# Autodesk Inventor assembly: Donna-Sym2
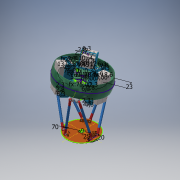
[picture p0: Inventor's stored thumbnail of the model, 180x180]
Saved by Autodesk Inventor 2018.2 (Build 222227000, 227)
## iProperties
Created: 2018-03-01
Part Number: Donna-Sym2
Material: Generisch
Document SubType Name: Assembly
Designer: JochenAlt
Author: JochenAlt
## Documents named in this file (5)
- D:\Projects\Donna\CAD\KST DS215MG\Donna-Sym.iam
- D:\Projects\Donna\CAD\KST DS215MG\Stewart-Sym-Base.iam
- D:\Projects\Donna\CAD\KST DS215MG\Body-Rod-KST215MG.iam
- D:\Projects\Donna\CAD\KST DS215MG\Servo-Arm-20mm-Enhanced-Ball-Joint.iam
- D:\Projects\Donna\CAD\KST DS215MG\Stewart-Body-Sym.iam
## Components (14 placed, 4 different names)
1. Stewart-Sym-Base:1 [sub-assembly] — Passend:1, Passend:2, Passend:3, Passend:4, Passend:5, Passend:6, Passend:7, Passend:8, Passend:9
2. BodyRod-KST215MG:1 [sub-assembly] — Passend:4, Passend:15
3. BodyRod-KST215MG:2 [sub-assembly] — Passend:5, Passend:12
4. BodyRod-KST215MG:3 [sub-assembly] — Passend:6, Passend:27
5. BodyRod-KST215MG:4 [sub-assembly] — Passend:7, Passend:24
6. BodyRod-KST215MG:5 [sub-assembly] — Passend:8, Passend:21
7. BodyRod-KST215MG:6 [sub-assembly] — Passend:9, Passend:18
8. Servo-Arm-20mm-Enhanced-Ball-Joint:1 [sub-assembly] — Passend:22, Passend:23, Passend:24
9. Servo-Arm-20mm-Enhanced-Ball-Joint:2 [sub-assembly] — Passend:10, Passend:11, Passend:12
10. Servo-Arm-20mm-Enhanced-Ball-Joint:3 [sub-assembly] — Passend:19, Passend:20, Passend:21
11. Servo-Arm-20mm-Enhanced-Ball-Joint:4 [sub-assembly] — Passend:25, Passend:26, Passend:27
12. Servo-Arm-20mm-Enhanced-Ball-Joint:5 [sub-assembly] — Passend:16, Passend:17, Passend:18
13. Servo-Arm-20mm-Enhanced-Ball-Joint:6 [sub-assembly] — Passend:13, Passend:14, Passend:15
14. Stewart-Bosy-Sym:1 [sub-assembly] — Passend:10, Passend:11, Passend:13, Passend:14, Passend:16, Passend:17, Passend:19, Passend:20, Passend:22, Passend:23, Passend:25, Passend:26
## Relationships (27: Mate 27)
- Passend:1 [Mate]: Stewart-Sym-Base:1
- Passend:2 [Mate]: Stewart-Sym-Base:1
- Passend:3 [Mate]: Stewart-Sym-Base:1
- Passend:4 [Mate]: Stewart-Sym-Base:1 ↔ BodyRod-KST215MG:1
- Passend:5 [Mate]: Stewart-Sym-Base:1 ↔ BodyRod-KST215MG:2
- Passend:6 [Mate]: Stewart-Sym-Base:1 ↔ BodyRod-KST215MG:3
- Passend:7 [Mate]: Stewart-Sym-Base:1 ↔ BodyRod-KST215MG:4
- Passend:8 [Mate]: Stewart-Sym-Base:1 ↔ BodyRod-KST215MG:5
- Passend:9 [Mate]: Stewart-Sym-Base:1 ↔ BodyRod-KST215MG:6
- Passend:10 [Mate]: Servo-Arm-20mm-Enhanced-Ball-Joint:2 ↔ Stewart-Bosy-Sym:1
- Passend:11 [Mate]: Servo-Arm-20mm-Enhanced-Ball-Joint:2 ↔ Stewart-Bosy-Sym:1
- Passend:12 [Mate]: BodyRod-KST215MG:2 ↔ Servo-Arm-20mm-Enhanced-Ball-Joint:2
- Passend:13 [Mate]: Servo-Arm-20mm-Enhanced-Ball-Joint:6 ↔ Stewart-Bosy-Sym:1
- Passend:14 [Mate]: Servo-Arm-20mm-Enhanced-Ball-Joint:6 ↔ Stewart-Bosy-Sym:1
- Passend:15 [Mate]: BodyRod-KST215MG:1 ↔ Servo-Arm-20mm-Enhanced-Ball-Joint:6
- Passend:16 [Mate]: Servo-Arm-20mm-Enhanced-Ball-Joint:5 ↔ Stewart-Bosy-Sym:1
- Passend:17 [Mate]: Servo-Arm-20mm-Enhanced-Ball-Joint:5 ↔ Stewart-Bosy-Sym:1
- Passend:18 [Mate]: BodyRod-KST215MG:6 ↔ Servo-Arm-20mm-Enhanced-Ball-Joint:5
- Passend:19 [Mate]: Servo-Arm-20mm-Enhanced-Ball-Joint:3 ↔ Stewart-Bosy-Sym:1
- Passend:20 [Mate]: Servo-Arm-20mm-Enhanced-Ball-Joint:3 ↔ Stewart-Bosy-Sym:1
- Passend:21 [Mate]: BodyRod-KST215MG:5 ↔ Servo-Arm-20mm-Enhanced-Ball-Joint:3
- Passend:22 [Mate]: Servo-Arm-20mm-Enhanced-Ball-Joint:1 ↔ Stewart-Bosy-Sym:1
- Passend:23 [Mate]: Servo-Arm-20mm-Enhanced-Ball-Joint:1 ↔ Stewart-Bosy-Sym:1
- Passend:24 [Mate]: BodyRod-KST215MG:4 ↔ Servo-Arm-20mm-Enhanced-Ball-Joint:1
- Passend:25 [Mate]: Servo-Arm-20mm-Enhanced-Ball-Joint:4 ↔ Stewart-Bosy-Sym:1
- Passend:26 [Mate]: Servo-Arm-20mm-Enhanced-Ball-Joint:4 ↔ Stewart-Bosy-Sym:1
- Passend:27 [Mate]: BodyRod-KST215MG:3 ↔ Servo-Arm-20mm-Enhanced-Ball-Joint:4
